# Autodesk Inventor assembly: s-assy-frame-connector
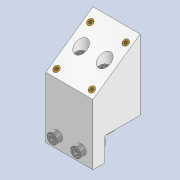
[picture p0: Inventor's stored thumbnail of the model, 180x180]
Saved by Autodesk Inventor 2022 (Build 260153000, 153)
## iProperties
Created: 2021-09-21
Part Number: s-assy-frame-connector
Document SubType Name: Assembly
Designer: yuto6
Mass: 104.335 g
Surface Area: 195.287 cm^2
Volume: 86.8438 cm^3
Density: 1.20141 g/cm^3
Author: yuto6
## Documents named in this file (6)
- C:\Users\yuta0\Documents\GitHub\catchrobo_hardware\assy-shooter\s-assy-frame-connector.iam
- C:\Users\yuta0\Documents\GitHub\catchrobo_hardware\assy-shooter\shooter_base2.ipt
- C:\Users\yuta0\Documents\GitHub\catchrobo_hardware\assy-shooter\SB-305060.ipt
- C:\Users\yuta0\Documents\GitHub\catchrobo_hardware\assy-shooter\CB5_40.ipt
- C:\Users\yuta0\Documents\GitHub\catchrobo_hardware\assy-shooter\CB5-15.ipt
- C:\Users\yuta0\Documents\GitHub\catchrobo_hardware\assy-shooter\HNTT5-5.ipt
## Components (15 placed, 5 different names)
1. shooter_base2:1 — メイト:7, フラッシュ:3, メイト:10, メイト:11, メイト:14, メイト:17, 角度:1, メイト:24, メイト:25, 角度:2, メイト:26, メイト:27, フラッシュ:4, フラッシュ:5
2. SB-305060:5 — メイト:26, フラッシュ:4
3. SB-305060:6 — メイト:27, フラッシュ:5
4. SB-305060:1 — メイト:7, フラッシュ:3
5. SB-305060:2
6. SB-305060:3
7. SB-305060:4
8. HNTT5-5:1 — メイト:22, 角度:1, メイト:25
9. CB5-15:1 — メイト:14, メイト:17, メイト:22
10. HNTT5-5:2 — メイト:23, メイト:24, 角度:2
11. CB5_40:1 — メイト:10, メイト:11, メイト:23
12. HNTT5-5:3
13. CB5-15:2
14. HNTT5-5:4
15. CB5_40:2
## Component patterns: (4 elements, first: SB-305060:1), (2 elements, first: HNTT5-5:1 + CB5-15:1 + HNTT5-5:2 + CB5_40:1)
## Relationships (16: Mate 11, Flush 3, Angle 2)
- メイト:7 [Mate]: shooter_base2:1 ↔ SB-305060:1
- フラッシュ:3 [Flush]: shooter_base2:1 ↔ SB-305060:1
- メイト:10 [Mate]: shooter_base2:1 ↔ CB5_40:1
- メイト:11 [Mate]: shooter_base2:1 ↔ CB5_40:1
- メイト:14 [Mate]: shooter_base2:1 ↔ CB5-15:1
- メイト:17 [Mate]: shooter_base2:1 ↔ CB5-15:1
- メイト:22 [Mate]: HNTT5-5:1 ↔ CB5-15:1
- 角度:1 [Angle] (0 deg): shooter_base2:1 ↔ HNTT5-5:1
- メイト:23 [Mate]: HNTT5-5:2 ↔ CB5_40:1
- メイト:24 [Mate] (2 mm): shooter_base2:1 ↔ HNTT5-5:2
- メイト:25 [Mate] (2 mm): shooter_base2:1 ↔ HNTT5-5:1
- 角度:2 [Angle] (0 deg): shooter_base2:1 ↔ HNTT5-5:2
- メイト:26 [Mate]: shooter_base2:1 ↔ SB-305060:5
- メイト:27 [Mate]: shooter_base2:1 ↔ SB-305060:6
- フラッシュ:4 [Flush]: shooter_base2:1 ↔ SB-305060:5
- フラッシュ:5 [Flush]: shooter_base2:1 ↔ SB-305060:6
